# Autodesk Inventor assembly: mechanum
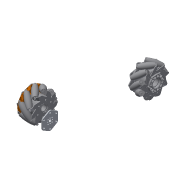
[picture p0: Inventor's stored thumbnail of the model, 180x180]
Saved by Autodesk Inventor 2018 (Build 220112000, 112)
## iProperties
Created: 2018-05-15
Part Number: mechanum
Document SubType Name: Assembly
Designer: ball
Author: ball
## Documents named in this file (4)
- C:\FTC\FTC8863CAD\2017Robot\mechanum.iam
- C:\FTC\FTC8863CAD\Andymark\am-2609a+FTC+Conversion+Plate+REV+2.ipt
- C:\FTC\FTC8863CAD\Andymark\4HD Mecanum Right.ipt
- C:\FTC\FTC8863CAD\Nexus-Wheels-STP\100mm Aluminum Mecanum wheels.ipt
## Components (3 placed, 3 different names)
1. am-2609a+FTC+Conversion+Plate+REV+2:1 — Mate:1
2. 4HD Mecanum Right:1
3. 100mm Aluminum Mecanum wheels:1 — Mate:1
## Relationships (1: Mate 1)
- Mate:1: am-2609a+FTC+Conversion+Plate+REV+2:1 ↔ 100mm Aluminum Mecanum wheels:1
